# Autodesk Inventor assembly: Charniere
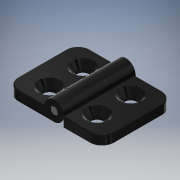
[picture p0: Inventor's stored thumbnail of the model, 180x180]
Saved by Autodesk Inventor 2017 (Build 210142000, 142)
## iProperties
Company: FABLAB Frecnhmakers
Part Number: Charniere
Project: 1400-PopCorn Machine
Material: Générique
Catalog Web Link: http://www.frenchmakers.com/
Document SubType Name: Assembly
Designer: FABLAB Frenchmakers
Stock Number: 1400-05-00
Author: Adrien MARY
## Documents named in this file (3)
- W:\Professionnel\Conception FABLAB\1400 Popcorn Machine\1400-05 Charniere\1400-05-00 Charniere.iam
- W:\Professionnel\Conception FABLAB\1400 Popcorn Machine\1400-05 Charniere\1400-05-01 Charnière A.ipt
- W:\Professionnel\Conception FABLAB\1400 Popcorn Machine\1400-05 Charniere\1400-05-03 Axe charniere.ipt
## Components (3 placed, 2 different names)
1. 1400-05-01 Charnière A:1 — Placage:5, Placage:6, Angle:1
2. 1400-05-03 Axe charniere:1 — Placage:4, Placage:5, Placage:7
3. 1400-05-01 Charnière A:2 — Placage:6, Placage:7, Angle:1
## Relationships (5: Mate 4, Angle 1)
- Placage:4 [Mate]: 1400-05-03 Axe charniere:1
- Placage:5 [Mate]: 1400-05-01 Charnière A:1 ↔ 1400-05-03 Axe charniere:1
- Placage:6 [Mate]: 1400-05-01 Charnière A:1 ↔ 1400-05-01 Charnière A:2
- Placage:7 [Mate]: 1400-05-03 Axe charniere:1 ↔ 1400-05-01 Charnière A:2
- Angle:1 (0 deg): 1400-05-01 Charnière A:1 ↔ 1400-05-01 Charnière A:2
